# Autodesk Inventor assembly: OurWheelAssemblyBig
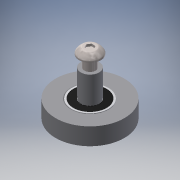
[picture p0: Inventor's stored thumbnail of the model, 180x180]
Saved by Autodesk Inventor 2017 (Build 210142000, 142)
## iProperties
Created: 2017-03-29
Part Number: OurWheelAssemblyBig
Document SubType Name: Assembly
Designer: umr
Author: umr
## Documents named in this file (6)
- D:\SeniorProject\Models2\WheelAssembly\OurWheelAssemblyBig.iam
- D:\SeniorProject\Models2\WheelAssembly\Precision Ball Bearing.ipt
- D:\SeniorProject\Models2\WheelAssembly\M5 Screw_30mm.ipt
- D:\SeniorProject\Models2\WheelAssembly\M5 Nut.ipt
- D:\SeniorProject\Models2\WheelAssembly\egzantrikNut.ipt
- D:\SeniorProject\Models2\WheelAssembly\Wheel_16-30.ipt
## Components (5 placed, 5 different names)
1. Precision Ball Bearing:1 — Mate:2, Mate:4, Mate:6, Mate:8, Mate:9
2. M5 Screw_30mm:1 — Mate:2, Mate:3, Mate:5, Mate:7
3. M5 Nut:1 — Mate:3, Mate:4
4. egzantrikNut:2 — Mate:5, Mate:6, Mate:7
5. Wheel_16-30:1 — Mate:8, Mate:9
## Relationships (8: Mate 8)
- Mate:2: Precision Ball Bearing:1 ↔ M5 Screw_30mm:1
- Mate:3: M5 Screw_30mm:1 ↔ M5 Nut:1
- Mate:4: Precision Ball Bearing:1 ↔ M5 Nut:1
- Mate:5: M5 Screw_30mm:1 ↔ egzantrikNut:2
- Mate:6: Precision Ball Bearing:1 ↔ egzantrikNut:2
- Mate:7 (5 mm): M5 Screw_30mm:1 ↔ egzantrikNut:2
- Mate:8: Precision Ball Bearing:1 ↔ Wheel_16-30:1
- Mate:9: Precision Ball Bearing:1 ↔ Wheel_16-30:1
